# Autodesk Inventor assembly: 歯付きベルト伝達
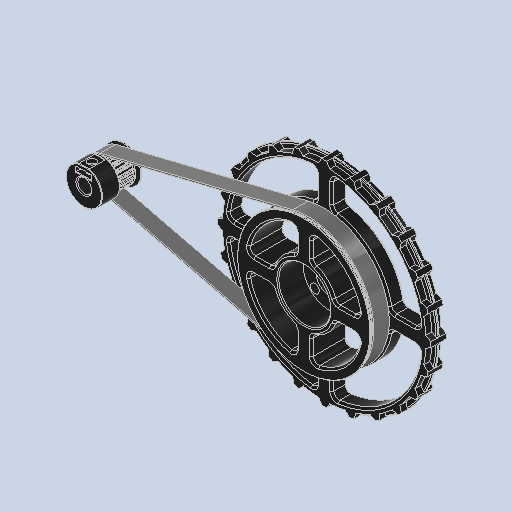
[picture p0: Inventor's stored thumbnail of the model, 512x512]
Saved by Autodesk Inventor 2025 (Build 290162000, 162)
## iProperties
ClientObjectVersion: 1
Created: 2024-06-24
Part Number: 歯付きベルト伝達
Document SubType Name: Assembly
Designer: 8326d
Author: 8326d
## Documents named in this file (4)
- C:\Users\8326d\Documents\hobby\CAD\General-Purpose-Robot\Pully_T2.5_16-64\timing_belt_pully.iam
- C:\Users\8326d\Documents\hobby\CAD\General-Purpose-Robot\Pully_T2.5_16-64\belt_T2.5-290.ipt
- C:\Users\8326d\Documents\hobby\CAD\General-Purpose-Robot\Pully_T2.5_16-64\pully_T2.5-16.ipt
- C:\Users\8326d\Documents\hobby\CAD\General-Purpose-Robot\Pully_T2.5_16-64\pully_T2.5-64.ipt
## Components (3 placed, 3 different names)
1. 歯付きベルト:1 — フラッシュ:1, メイト:1, メイト:2, フラッシュ:2, メイト:3, メイト:4
2. 歯付きプーリ1:1 — フラッシュ:1, メイト:1, メイト:2, 回転:1
3. 歯付きプーリ2:1 — フラッシュ:2, メイト:3, 回転:1, メイト:4
## Relationships (7: Mate 4, Flush 2, RelateRotation 1)
- フラッシュ:1 [Flush]: 歯付きベルト:1 ↔ 歯付きプーリ1:1
- メイト:1 [Mate]: 歯付きベルト:1 ↔ 歯付きプーリ1:1
- メイト:2 [Mate]: 歯付きベルト:1 ↔ 歯付きプーリ1:1
- フラッシュ:2 [Flush]: 歯付きベルト:1 ↔ 歯付きプーリ2:1
- メイト:3 [Mate]: 歯付きベルト:1 ↔ 歯付きプーリ2:1
- 回転:1 [RelateRotation] (4 ul): 歯付きプーリ1:1 ↔ 歯付きプーリ2:1
- メイト:4 [Mate]: 歯付きベルト:1 ↔ 歯付きプーリ2:1
